# Autodesk Inventor assembly: bat_mount_v2
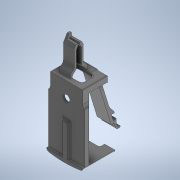
[picture p0: Inventor's stored thumbnail of the model, 180x180]
Saved by Autodesk Inventor 2020 (Build 240168000, 168)
## iProperties
Created: 2024-03-27
Part Number: bat_mount_v2
Document SubType Name: Assembly
Designer: 4s
Author: 4s
## Documents named in this file (3)
- C:\Users\4s\Documents\Inventor models\Asterisk\robot_v2\Bat_mount\bat_mount_v2.iam
- C:\Users\4s\Documents\Inventor models\Asterisk\robot_v2\Bat_mount\bat_case_v5.ipt
- C:\Users\4s\Documents\Inventor models\Asterisk\robot_v2\Bat_mount\bat_lock03.ipt
## Components (2 placed, 2 different names)
1. bat_case_v5:1 — Совмещение:1, Заподлицо:1, Совмещение:2, Заподлицо:2, Совмещение:3, Заподлицо:3
2. bat_lock03:1 — Совмещение:1, Заподлицо:1, Заподлицо:3
## Relationships (6: Mate 3, Flush 3)
- Совмещение:1 [Mate] (-5 mm): bat_case_v5:1 ↔ bat_lock03:1
- Заподлицо:1 [Flush] (12 mm): bat_case_v5:1 ↔ bat_lock03:1
- Совмещение:2 [Mate]: bat_case_v5:1
- Заподлицо:2 [Flush]: bat_case_v5:1
- Совмещение:3 [Mate]: bat_case_v5:1
- Заподлицо:3 [Flush]: bat_case_v5:1 ↔ bat_lock03:1
